# Autodesk Inventor assembly: RadLWL
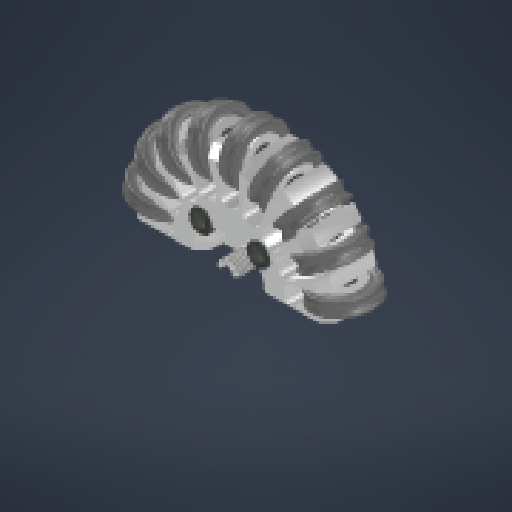
[picture p0: Inventor's stored thumbnail of the model, 512x512]
Saved by Autodesk Inventor 2026.1 (Build 301233020, 233B)
## iProperties
Created: 2025-03-24
Part Number: RadLWL
Document SubType Name: Assembly
Designer: Faabs
Author: Faabs
## Documents named in this file (7)
- C:\Users\Bahaa\Nextcloud2\CAD\25-26\RadLWL\RadLWL.iam
- C:\Users\Bahaa\Nextcloud2\CAD\25-26\RadLWL\Radkasten.ipt
- C:\Users\Bahaa\Nextcloud2\CAD\25-26\RadLWL\Rolle\UBG-Rolle.iam
- C:\Users\Bahaa\Nextcloud2\CAD\25-26\RadLWL\Raddeckel.ipt
- C:\Users\Bahaa\Nextcloud2\CAD\25-26\RadLWL\DIN 912 - M3 x 0,5 x 6 x 4,75.ipt
- C:\Users\JurijLenz\Documents\Inventor\Content Center Files\R2026\de-DE\AS 1474(1)\AS 1474 - M5(1).ipt
- C:\Users\Bahaa\Nextcloud2\CAD\25-26\RadLWL\Radadapter.ipt
## Components (26 placed, 6 different names)
1. Radkasten:1 — Flush:1, Flush:2, Flush:3, Mate:1, Mate:2, Mate:4, Mate:5, Mate:7, Mate:8, Mate:14, Mate:15, Mate:16, Angle:1
2. Raddeckel:1 — Mate:4, Mate:5, Mate:8, Insert:1, Insert:2, Insert:3, Insert:4
3. AS 1474 - Metrisch M5:1 — Mate:14, Mate:17
4. Radadapter:1 — Mate:15, Mate:16, Angle:1, Mate:17
5. DIN 912 - ersetzt durch DIN EN ISO 4762 M3 x 6:4 — Insert:1
6. DIN 912 - ersetzt durch DIN EN ISO 4762 M3 x 6:3 — Insert:3
7. DIN 912 - ersetzt durch DIN EN ISO 4762 M3 x 6:2 — Insert:4
8. DIN 912 - ersetzt durch DIN EN ISO 4762 M3 x 6:1 — Insert:2
9. UBG-Rolle:1 [sub-assembly] — Mate:1, Mate:2, Mate:7
10. UBG-Rolle:2 [sub-assembly]
11. UBG-Rolle:3 [sub-assembly]
12. UBG-Rolle:4 [sub-assembly]
13. UBG-Rolle:5 [sub-assembly]
14. UBG-Rolle:6 [sub-assembly]
15. UBG-Rolle:7 [sub-assembly]
16. UBG-Rolle:8 [sub-assembly]
17. UBG-Rolle:9 [sub-assembly]
18. UBG-Rolle:10 [sub-assembly]
19. UBG-Rolle:11 [sub-assembly]
20. UBG-Rolle:12 [sub-assembly]
21. UBG-Rolle:13 [sub-assembly]
22. UBG-Rolle:14 [sub-assembly]
23. UBG-Rolle:15 [sub-assembly]
24. UBG-Rolle:16 [sub-assembly]
25. UBG-Rolle:17 [sub-assembly]
26. UBG-Rolle:18 [sub-assembly]
## Component patterns: (18 elements, first: UBG-Rolle:1)
## Relationships (18: Mate 10, Insert 4, Flush 3, Angle 1)
- Flush:1: Radkasten:1
- Flush:2: Radkasten:1
- Flush:3: Radkasten:1
- Mate:1: Radkasten:1 ↔ UBG-Rolle:1
- Mate:2 (0.2 mm): Radkasten:1 ↔ UBG-Rolle:1
- Mate:4: Radkasten:1 ↔ Raddeckel:1
- Mate:5: Radkasten:1 ↔ Raddeckel:1
- Mate:7 (7 mm): Radkasten:1 ↔ UBG-Rolle:1
- Mate:8: Radkasten:1 ↔ Raddeckel:1
- Insert:1: Raddeckel:1 ↔ DIN 912 - ersetzt durch DIN EN ISO 4762 M3 x 6:4
- Insert:2: Raddeckel:1 ↔ DIN 912 - ersetzt durch DIN EN ISO 4762 M3 x 6:1
- Insert:3: Raddeckel:1 ↔ DIN 912 - ersetzt durch DIN EN ISO 4762 M3 x 6:3
- Insert:4: Raddeckel:1 ↔ DIN 912 - ersetzt durch DIN EN ISO 4762 M3 x 6:2
- Mate:14: Radkasten:1 ↔ AS 1474 - Metrisch M5:1
- Mate:15: Radkasten:1 ↔ Radadapter:1
- Mate:16: Radkasten:1 ↔ Radadapter:1
- Angle:1 (0 deg): Radkasten:1 ↔ Radadapter:1
- Mate:17: AS 1474 - Metrisch M5:1 ↔ Radadapter:1
